# Autodesk Inventor assembly: Ensamblaje_Robot_Semillero
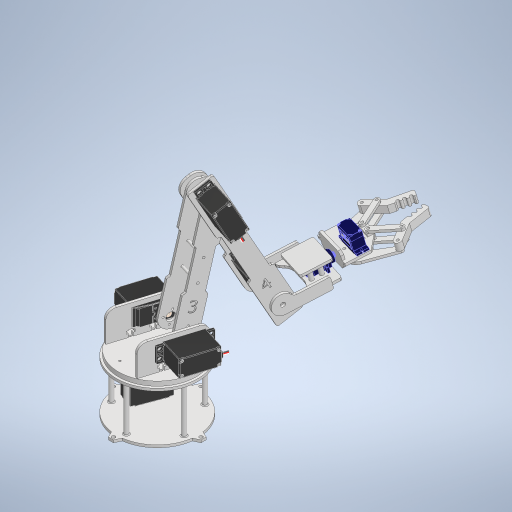
[picture p0: Inventor's stored thumbnail of the model, 512x512]
Saved by Autodesk Inventor 2023 (Build 270158000, 158)
## iProperties
Created: 2024-09-27
Part Number: Ensamblaje_Robot_Semillero
Document SubType Name: Assembly
Designer: sebas
Author: sebas
## Documents named in this file (12)
- C:\Users\sebas\OneDrive\Documentos\ILLERO_MODELADO_ROBOT\Ensamblaje_Robot_Semillero.iam
- C:\Users\sebas\OneDrive\Documentos\ILLERO_MODELADO_ROBOT\Pieza_base_1.ipt
- C:\Users\sebas\OneDrive\Documentos\ILLERO_MODELADO_ROBOT\Pieza_base_2.ipt
- C:\Users\sebas\OneDrive\Documentos\ILLERO_MODELADO_ROBOT\Pieza_eslabon_3.ipt
- C:\Users\sebas\OneDrive\Documentos\ILLERO_MODELADO_ROBOT\Pieza_eslabon_4.ipt
- C:\Users\sebas\OneDrive\Documentos\ILLERO_MODELADO_ROBOT\Pieza_5.ipt
- C:\Users\sebas\OneDrive\Documentos\ILLERO_MODELADO_ROBOT\User Library-Subasa Servo S3003.ipt
- C:\Users\sebas\OneDrive\Documentos\ILLERO_MODELADO_ROBOT\MicroServo-SG90.ipt
- C:\Users\sebas\OneDrive\Documentos\ILLERO_MODELADO_ROBOT\Pinza_pieza1.ipt
- C:\Users\sebas\OneDrive\Documentos\ILLERO_MODELADO_ROBOT\Pinza_pieza2.ipt
- C:\Users\sebas\OneDrive\Documentos\ILLERO_MODELADO_ROBOT\Pinza_pieza3.ipt
- C:\Users\sebas\OneDrive\Documentos\ILLERO_MODELADO_ROBOT\Pinza_pieza4.ipt
## Components (21 placed, 11 different names)
1. Pieza_base_1:1 — Coincidencia:3, Coincidencia:4, Coincidencia:17
2. Pieza_base_2:1 — Coincidencia:3, Coincidencia:4, Coincidencia:6, Coincidencia:18, Coincidencia:19, Coincidencia:20, Coincidencia:21, Coincidencia:22, Coincidencia:23, Coincidencia:24
3. Pieza_eslabon_3:1 — Coincidencia:6, Coincidencia:7, Coincidencia:28, Coincidencia:33
4. Pieza_eslabon_4:1 — Coincidencia:7, Coincidencia:9, Coincidencia:25, Coincidencia:26, Coincidencia:27, Coincidencia:29, Coincidencia:30, Coincidencia:31
5. Pieza_5:1 — Coincidencia:9, Coincidencia:32, Coincidencia:34, Nivelación:1, Nivelación:2
6. User Library-Subasa Servo S3003:1 — Coincidencia:19, Coincidencia:20, Coincidencia:21
7. User Library-Subasa Servo S3003:3 — Coincidencia:25, Coincidencia:26, Coincidencia:27, Coincidencia:28
8. User Library-Subasa Servo S3003:4 — Coincidencia:17, Coincidencia:18
9. User Library-Subasa Servo S3003:5 — Coincidencia:22, Coincidencia:23, Coincidencia:24, Coincidencia:33
10. User Library-Subasa Servo S3003:6 — Coincidencia:29, Coincidencia:30, Coincidencia:31, Coincidencia:32
11. MicroServo-SG90:1 — Coincidencia:34, Nivelación:1, Nivelación:2, Coincidencia:35, Coincidencia:37
12. Pinza_pieza1:1 — Coincidencia:35, Coincidencia:37, Coincidencia:38, Coincidencia:39, Coincidencia:40, Coincidencia:41, Coincidencia:42, Coincidencia:43, Coincidencia:44, Coincidencia:45, Coincidencia:52, Coincidencia:59, Coincidencia:60, Coincidencia:62, Coincidencia:63
13. Pinza_pieza2:1 — Coincidencia:38, Coincidencia:39, Coincidencia:48, Coincidencia:49
14. Pinza_pieza2:2 — Coincidencia:40, Coincidencia:41, Coincidencia:46, Coincidencia:47
15. Pinza_pieza2:3 — Coincidencia:42, Coincidencia:43, Coincidencia:58
16. Pinza_pieza2:4 — Coincidencia:44, Coincidencia:45, Coincidencia:50
17. Pinza_pieza3:2 — Coincidencia:46, Coincidencia:47, Coincidencia:50, Coincidencia:64
18. Pinza_pieza3:3 — Coincidencia:48, Coincidencia:49, Coincidencia:56, Coincidencia:57, Coincidencia:58
19. MicroServo-SG90:2 — Coincidencia:52, Coincidencia:59, Coincidencia:60, Coincidencia:61
20. Pinza_pieza4:1 — Coincidencia:56, Coincidencia:57, Coincidencia:61
21. Pinza_pieza4:2 — Coincidencia:62, Coincidencia:63, Coincidencia:64
## Relationships (50: Mate 48, Flush 2)
- Coincidencia:3 [Mate]: Pieza_base_1:1 ↔ Pieza_base_2:1
- Coincidencia:4 [Mate] (0.5 mm): Pieza_base_1:1 ↔ Pieza_base_2:1
- Coincidencia:6 [Mate] (11 mm): Pieza_base_2:1 ↔ Pieza_eslabon_3:1
- Coincidencia:7 [Mate] (5 mm): Pieza_eslabon_3:1 ↔ Pieza_eslabon_4:1
- Coincidencia:9 [Mate] (4 mm): Pieza_eslabon_4:1 ↔ Pieza_5:1
- Coincidencia:17 [Mate]: Pieza_base_1:1 ↔ User Library-Subasa Servo S3003:4
- Coincidencia:18 [Mate]: Pieza_base_2:1 ↔ User Library-Subasa Servo S3003:4
- Coincidencia:19 [Mate]: Pieza_base_2:1 ↔ User Library-Subasa Servo S3003:1
- Coincidencia:20 [Mate]: Pieza_base_2:1 ↔ User Library-Subasa Servo S3003:1
- Coincidencia:21 [Mate]: Pieza_base_2:1 ↔ User Library-Subasa Servo S3003:1
- Coincidencia:22 [Mate]: Pieza_base_2:1 ↔ User Library-Subasa Servo S3003:5
- Coincidencia:23 [Mate]: Pieza_base_2:1 ↔ User Library-Subasa Servo S3003:5
- Coincidencia:24 [Mate]: Pieza_base_2:1 ↔ User Library-Subasa Servo S3003:5
- Coincidencia:25 [Mate]: Pieza_eslabon_4:1 ↔ User Library-Subasa Servo S3003:3
- Coincidencia:26 [Mate]: Pieza_eslabon_4:1 ↔ User Library-Subasa Servo S3003:3
- Coincidencia:27 [Mate]: Pieza_eslabon_4:1 ↔ User Library-Subasa Servo S3003:3
- Coincidencia:28 [Mate]: Pieza_eslabon_3:1 ↔ User Library-Subasa Servo S3003:3
- Coincidencia:29 [Mate]: Pieza_eslabon_4:1 ↔ User Library-Subasa Servo S3003:6
- Coincidencia:30 [Mate]: Pieza_eslabon_4:1 ↔ User Library-Subasa Servo S3003:6
- Coincidencia:31 [Mate]: Pieza_eslabon_4:1 ↔ User Library-Subasa Servo S3003:6
- Coincidencia:32 [Mate]: Pieza_5:1 ↔ User Library-Subasa Servo S3003:6
- Coincidencia:33 [Mate]: Pieza_eslabon_3:1 ↔ User Library-Subasa Servo S3003:5
- Coincidencia:34 [Mate]: Pieza_5:1 ↔ MicroServo-SG90:1
- Nivelación:1 [Flush]: Pieza_5:1 ↔ MicroServo-SG90:1
- Nivelación:2 [Flush]: Pieza_5:1 ↔ MicroServo-SG90:1
- Coincidencia:35 [Mate]: MicroServo-SG90:1 ↔ Pinza_pieza1:1
- Coincidencia:37 [Mate]: MicroServo-SG90:1 ↔ Pinza_pieza1:1
- Coincidencia:38 [Mate]: Pinza_pieza1:1 ↔ Pinza_pieza2:1
- Coincidencia:39 [Mate]: Pinza_pieza1:1 ↔ Pinza_pieza2:1
- Coincidencia:40 [Mate]: Pinza_pieza1:1 ↔ Pinza_pieza2:2
- Coincidencia:41 [Mate]: Pinza_pieza1:1 ↔ Pinza_pieza2:2
- Coincidencia:42 [Mate]: Pinza_pieza1:1 ↔ Pinza_pieza2:3
- Coincidencia:43 [Mate]: Pinza_pieza1:1 ↔ Pinza_pieza2:3
- Coincidencia:44 [Mate]: Pinza_pieza1:1 ↔ Pinza_pieza2:4
- Coincidencia:45 [Mate]: Pinza_pieza1:1 ↔ Pinza_pieza2:4
- Coincidencia:46 [Mate]: Pinza_pieza2:2 ↔ Pinza_pieza3:2
- Coincidencia:47 [Mate]: Pinza_pieza2:2 ↔ Pinza_pieza3:2
- Coincidencia:48 [Mate]: Pinza_pieza2:1 ↔ Pinza_pieza3:3
- Coincidencia:49 [Mate]: Pinza_pieza2:1 ↔ Pinza_pieza3:3
- Coincidencia:50 [Mate]: Pinza_pieza2:4 ↔ Pinza_pieza3:2
- Coincidencia:52 [Mate]: Pinza_pieza1:1 ↔ MicroServo-SG90:2
- Coincidencia:56 [Mate]: Pinza_pieza3:3 ↔ Pinza_pieza4:1
- Coincidencia:57 [Mate]: Pinza_pieza3:3 ↔ Pinza_pieza4:1
- Coincidencia:58 [Mate]: Pinza_pieza2:3 ↔ Pinza_pieza3:3
- Coincidencia:59 [Mate]: Pinza_pieza1:1 ↔ MicroServo-SG90:2
- Coincidencia:60 [Mate]: Pinza_pieza1:1 ↔ MicroServo-SG90:2
- Coincidencia:61 [Mate]: MicroServo-SG90:2 ↔ Pinza_pieza4:1
- Coincidencia:62 [Mate] (3 mm): Pinza_pieza1:1 ↔ Pinza_pieza4:2
- Coincidencia:63 [Mate]: Pinza_pieza1:1 ↔ Pinza_pieza4:2
- Coincidencia:64 [Mate]: Pinza_pieza3:2 ↔ Pinza_pieza4:2
